# Autodesk Inventor assembly: MasterAssem-Chassis
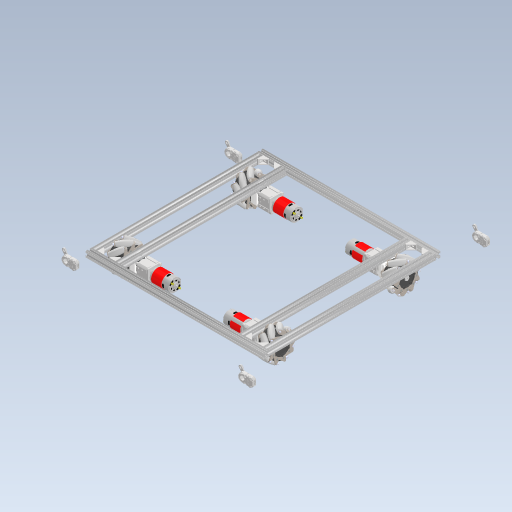
[picture p0: Inventor's stored thumbnail of the model, 512x512]
Saved by Autodesk Inventor 2023 (Build 270158000, 158)
## iProperties
Created: 2022-07-11
Part Number: MasterAssem-Chassis
Document SubType Name: Assembly
Designer: Dave
Author: Dave
## Documents named in this file (5)
- C:\Users\Dave\Documents\GrabCAD\Chalk Bot\Chalkbot1.0\Chassis\V1\MasterAssem-Chassis.iam
- C:\Users\Dave\Documents\GrabCAD\Chalk Bot\Chalkbot1.0\Chassis\V1\ChassisFrame-SubAssem01.iam
- C:\Users\Dave\Documents\GrabCAD\Chalk Bot\Chalkbot1.0\Chassis\V1\LeftMecanum-SubAssem01.iam
- C:\Users\Dave\Documents\GrabCAD\Chalk Bot\Chalkbot1.0\Chassis\V1\RightMecanum-SubAssem01.iam
- C:\Users\Dave\Documents\GrabCAD\Chalk Bot\Chalkbot1.0\Chassis\V1\Encoder Step Files\REV-11-1271.ipt
## Components (9 placed, 4 different names)
1. ChassisFrame-SubAssem01:1 [sub-assembly] — Mate:3, Mate:4, Mate:5, Mate:6, Mate:7, Mate:8, Mate:11, Mate:12
2. LeftMecanum-SubAssem01:1 [sub-assembly] — Mate:4, Mate:7, Mate:9
3. RightMecanum-SubAssem01:1 [sub-assembly] — Mate:3, Mate:8, Mate:10, Flush:1
4. RightMecanum-SubAssem01:2 [sub-assembly] — Mate:5, Mate:9, Flush:2, Mate:11
5. LeftMecanum-SubAssem01:2 [sub-assembly] — Mate:6, Mate:10, Flush:1, Flush:2, Mate:12
6. REV-11-1271:1
7. REV-11-1271:2
8. REV-11-1271:3
9. REV-11-1271:4
## Relationships (12: Mate 10, Flush 2)
- Mate:3: ChassisFrame-SubAssem01:1 ↔ RightMecanum-SubAssem01:1
- Mate:4: ChassisFrame-SubAssem01:1 ↔ LeftMecanum-SubAssem01:1
- Mate:5 (5 mm): ChassisFrame-SubAssem01:1 ↔ RightMecanum-SubAssem01:2
- Mate:6 (5 mm): ChassisFrame-SubAssem01:1 ↔ LeftMecanum-SubAssem01:2
- Mate:7 (5 mm): ChassisFrame-SubAssem01:1 ↔ LeftMecanum-SubAssem01:1
- Mate:8 (5 mm): ChassisFrame-SubAssem01:1 ↔ RightMecanum-SubAssem01:1
- Mate:9: LeftMecanum-SubAssem01:1 ↔ RightMecanum-SubAssem01:2
- Mate:10: RightMecanum-SubAssem01:1 ↔ LeftMecanum-SubAssem01:2
- Flush:1: RightMecanum-SubAssem01:1 ↔ LeftMecanum-SubAssem01:2
- Flush:2: RightMecanum-SubAssem01:2 ↔ LeftMecanum-SubAssem01:2
- Mate:11 (50 mm): ChassisFrame-SubAssem01:1 ↔ RightMecanum-SubAssem01:2
- Mate:12 (50 mm): ChassisFrame-SubAssem01:1 ↔ LeftMecanum-SubAssem01:2
